# Autodesk Inventor assembly: 000 Ensamblaje hw_LM - BASIC
(part 3 of 4)
- [Flush]: UND_0201CR___ _________:69 ↔ UND_0201CR___ _________:70
- [Flush]: UND_0201CR___ _________:75 ↔ UND_0201CR___ _________:77
- [Flush]: UND_0201CR___ _________:76 ↔ UND_0201CR___ _________:77
- [Flush]: UND_0201CR___ _________:74 ↔ UND_0201CR___ _________:77
- [Flush]: UND_0201CR___ _________:73 ↔ UND_0201CR___ _________:75
- [Flush]: UND_0201CR___ _________:71 ↔ UND_0201CR___ _________:74
- [Flush]: UND_0201CR___ _________:72 ↔ UND_0201CR___ _________:75
- Flush:768: UND_0201CR___ _________:44 ↔ UND_0201CR___ _________:51
- Flush:769: UND_0201CR___ _________:43 ↔ UND_0201CR___ _________:76
- Flush:770: UND_0201CR___ _________:49 ↔ UND_0201CR___ _________:57
- Flush:771: UND_0201CR___ _________:60 ↔ UND_0201CR___ _________:67
- Flush:772: UND_0201CR___ _________:8 ↔ UND_0201CR___ _________:40
- Flush:773: UND_0201CR___ _________:69 ↔ UND_0201CR___ _________:77
- [Flush]: UND_0201CR___ _________:79 ↔ UND_0201CR___ _________:82
- [Flush]: UND_0201CR___ _________:81 ↔ UND_0201CR___ _________:82
- [Flush]: UND_0201CR___ _________:78 ↔ UND_0201CR___ _________:82
- [Flush]: UND_0201CR___ _________:80 ↔ UND_0201CR___ _________:83
- [Flush]: UND_0201CR___ _________:79 ↔ UND_0201CR___ _________:80
- [Flush]: UND_0201CR___ _________:86 ↔ UND_0201CR___ _________:89
- [Flush]: UND_0201CR___ _________:88 ↔ UND_0201CR___ _________:89
- [Flush]: UND_0201CR___ _________:85 ↔ UND_0201CR___ _________:89
- [Flush]: UND_0201CR___ _________:87 ↔ UND_0201CR___ _________:90
- [Flush]: UND_0201CR___ _________:86 ↔ UND_0201CR___ _________:87
- [Flush]: UND_0201CR___ _________:92 ↔ UND_0201CR___ _________:94
- [Flush]: UND_0201CR___ _________:93 ↔ UND_0201CR___ _________:94
- [Flush]: UND_0201CR___ _________:91 ↔ UND_0201CR___ _________:94
- [Flush]: UND_0201CR___ _________:90 ↔ UND_0201CR___ _________:92
- [Flush]: UND_0201CR___ _________:88 ↔ UND_0201CR___ _________:91
- [Flush]: UND_0201CR___ _________:89 ↔ UND_0201CR___ _________:92
- [Flush]: UND_0201CR___ _________:78 ↔ UND_0201CR___ _________:84
- [Flush]: UND_0201CR___ _________:86 ↔ UND_0201CR___ _________:94
- Flush:792: UND_0201CR___ _________:64 ↔ UND_0201CR___ _________:82
- Flush:793: UND_0201CR___ _________:60 ↔ UND_0201CR___ _________:88
- Flush:794: UND_0201CR___ _________:50 ↔ UND_0201CR___ _________:84
- Flush:795: UND_0201CR___ _________:65 ↔ UND_0201CR___ _________:90
- Flush:796: UND_0201CR___ _________:67 ↔ UND_0201CR___ _________:92
- Flush:797: UND_0201CR___ _________:57 ↔ UND_0201CR___ _________:70
- Flush:798: UND_0201CR___ _________:6 ↔ UND_0201CR___ _________:67
- Flush:799: UND_0201CR___ _________:39 ↔ UND_0201CR___ _________:83
- [Flush]: UND_0201CR___ _________:96 ↔ UND_0201CR___ _________:99
- [Flush]: UND_0201CR___ _________:98 ↔ UND_0201CR___ _________:99
- [Flush]: UND_0201CR___ _________:95 ↔ UND_0201CR___ _________:99
- [Flush]: UND_0201CR___ _________:97 ↔ UND_0201CR___ _________:100
- [Flush]: UND_0201CR___ _________:96 ↔ UND_0201CR___ _________:97
- [Flush]: UND_0201CR___ _________:103 ↔ UND_0201CR___ _________:106
- [Flush]: UND_0201CR___ _________:105 ↔ UND_0201CR___ _________:106
- [Flush]: UND_0201CR___ _________:102 ↔ UND_0201CR___ _________:106
- [Flush]: UND_0201CR___ _________:104 ↔ UND_0201CR___ _________:107
- [Flush]: UND_0201CR___ _________:103 ↔ UND_0201CR___ _________:104
- [Flush]: UND_0201CR___ _________:109 ↔ UND_0201CR___ _________:111
- [Flush]: UND_0201CR___ _________:110 ↔ UND_0201CR___ _________:111
- [Flush]: UND_0201CR___ _________:108 ↔ UND_0201CR___ _________:111
- [Flush]: UND_0201CR___ _________:107 ↔ UND_0201CR___ _________:109
- [Flush]: UND_0201CR___ _________:105 ↔ UND_0201CR___ _________:108
- [Flush]: UND_0201CR___ _________:106 ↔ UND_0201CR___ _________:109
- [Flush]: UND_0201CR___ _________:95 ↔ UND_0201CR___ _________:101
- [Flush]: UND_0201CR___ _________:103 ↔ UND_0201CR___ _________:111
- Flush:818: UND_0201CR___ _________:92 ↔ UND_0201CR___ _________:108
- Flush:819: UND_0201CR___ _________:81 ↔ UND_0201CR___ _________:101
- [Flush]: UND_0201CR___ _________:112 ↔ UND_0201CR___ _________:113
- Angle:201 (0 deg): AQ24CANFD-02HTG:8 ↔ UND_0201CR___ _________:112
- Angle:202 (0 deg): UND_0201CR___ _________:112 ↔ UND_0201CR___ _________:114
- Angle:203 (0 deg): UND_0201CR___ _________:113 ↔ UND_0201CR___ _________:114
- Flush:821: UND_0201CR___ _________:113 ↔ UND_0201CR___ _________:114
- Flush:822: UND_0201CR___ _________:112 ↔ UND_0201CR___ _________:113
- Flush:823: UND_0201CR___ _________:84 ↔ UND_0201CR___ _________:113
- [Flush]: UND_0201CR___ _________:115 ↔ UND_0201CR___ _________:116
- [Angle] (0 deg): UND_0201CR___ _________:115 ↔ UND_0201CR___ _________:117
- [Angle] (0 deg): UND_0201CR___ _________:116 ↔ UND_0201CR___ _________:117
- [Flush]: UND_0201CR___ _________:116 ↔ UND_0201CR___ _________:117
- [Flush]: UND_0201CR___ _________:115 ↔ UND_0201CR___ _________:116
- [Flush]: UND_0201CR___ _________:118 ↔ UND_0201CR___ _________:119
- [Angle] (0 deg): UND_0201CR___ _________:118 ↔ UND_0201CR___ _________:120
- [Angle] (0 deg): UND_0201CR___ _________:119 ↔ UND_0201CR___ _________:120
- [Flush]: UND_0201CR___ _________:119 ↔ UND_0201CR___ _________:120
- [Flush]: UND_0201CR___ _________:118 ↔ UND_0201CR___ _________:119
- Flush:830: UND_0201CR___ _________:114 ↔ UND_0201CR___ _________:117
- Flush:831: UND_0201CR___ _________:112 ↔ UND_0201CR___ _________:118
- Flush:832: UND_0201CR___ _________:113 ↔ UND_0201CR___ _________:116
- Flush:833: UND_0201CR___ _________:115 ↔ UND_0201CR___ _________:118
- [Flush]: UND_0201CR___ _________:121 ↔ UND_0201CR___ _________:122
- [Angle] (0 deg): UND_0201CR___ _________:121 ↔ UND_0201CR___ _________:123
- [Angle] (0 deg): UND_0201CR___ _________:122 ↔ UND_0201CR___ _________:123
- [Flush]: UND_0201CR___ _________:122 ↔ UND_0201CR___ _________:123
- [Flush]: UND_0201CR___ _________:121 ↔ UND_0201CR___ _________:122
- [Flush]: UND_0201CR___ _________:124 ↔ UND_0201CR___ _________:125
- [Angle] (0 deg): UND_0201CR___ _________:124 ↔ UND_0201CR___ _________:126
- [Angle] (0 deg): UND_0201CR___ _________:125 ↔ UND_0201CR___ _________:126
- [Flush]: UND_0201CR___ _________:125 ↔ UND_0201CR___ _________:126
- [Flush]: UND_0201CR___ _________:124 ↔ UND_0201CR___ _________:125
- [Flush]: UND_0201CR___ _________:127 ↔ UND_0201CR___ _________:128
- [Angle] (0 deg): UND_0201CR___ _________:127 ↔ UND_0201CR___ _________:129
- [Angle] (0 deg): UND_0201CR___ _________:128 ↔ UND_0201CR___ _________:129
- [Flush]: UND_0201CR___ _________:128 ↔ UND_0201CR___ _________:129
- [Flush]: UND_0201CR___ _________:127 ↔ UND_0201CR___ _________:128
- [Flush]: UND_0201CR___ _________:123 ↔ UND_0201CR___ _________:126
- [Flush]: UND_0201CR___ _________:121 ↔ UND_0201CR___ _________:127
- [Flush]: UND_0201CR___ _________:122 ↔ UND_0201CR___ _________:125
- [Flush]: UND_0201CR___ _________:124 ↔ UND_0201CR___ _________:127
- [Flush]: UND_0201CR___ _________:130 ↔ UND_0201CR___ _________:131
- [Angle] (0 deg): UND_0201CR___ _________:130 ↔ UND_0201CR___ _________:132
- [Angle] (0 deg): UND_0201CR___ _________:131 ↔ UND_0201CR___ _________:132
- [Flush]: UND_0201CR___ _________:131 ↔ UND_0201CR___ _________:132
- [Flush]: UND_0201CR___ _________:130 ↔ UND_0201CR___ _________:131
- [Flush]: UND_0201CR___ _________:133 ↔ UND_0201CR___ _________:134
- [Angle] (0 deg): UND_0201CR___ _________:133 ↔ UND_0201CR___ _________:135
- [Angle] (0 deg): UND_0201CR___ _________:134 ↔ UND_0201CR___ _________:135
- [Flush]: UND_0201CR___ _________:134 ↔ UND_0201CR___ _________:135
- [Flush]: UND_0201CR___ _________:133 ↔ UND_0201CR___ _________:134
- [Flush]: UND_0201CR___ _________:136 ↔ UND_0201CR___ _________:137
- [Angle] (0 deg): UND_0201CR___ _________:136 ↔ UND_0201CR___ _________:138
- [Angle] (0 deg): UND_0201CR___ _________:137 ↔ UND_0201CR___ _________:138
- [Flush]: UND_0201CR___ _________:137 ↔ UND_0201CR___ _________:138
- [Flush]: UND_0201CR___ _________:136 ↔ UND_0201CR___ _________:137
- [Flush]: UND_0201CR___ _________:132 ↔ UND_0201CR___ _________:135
- [Flush]: UND_0201CR___ _________:130 ↔ UND_0201CR___ _________:136
- [Flush]: UND_0201CR___ _________:131 ↔ UND_0201CR___ _________:134
- [Flush]: UND_0201CR___ _________:133 ↔ UND_0201CR___ _________:136
- Flush:860: UND_0201CR___ _________:84 ↔ UND_0201CR___ _________:129
- Flush:861: UND_0201CR___ _________:122 ↔ UND_0201CR___ _________:132
- Flush:862: UND_0201CR___ _________:125 ↔ UND_0201CR___ _________:133
- [Flush]: UND_0201CR___ _________:139 ↔ UND_0201CR___ _________:140
- [Angle] (0 deg): UND_0201CR___ _________:139 ↔ UND_0201CR___ _________:141
- [Angle] (0 deg): UND_0201CR___ _________:140 ↔ UND_0201CR___ _________:141
- [Flush]: UND_0201CR___ _________:140 ↔ UND_0201CR___ _________:141
- [Flush]: UND_0201CR___ _________:139 ↔ UND_0201CR___ _________:140
- [Flush]: UND_0201CR___ _________:142 ↔ UND_0201CR___ _________:143
- [Angle] (0 deg): UND_0201CR___ _________:142 ↔ UND_0201CR___ _________:144
- [Angle] (0 deg): UND_0201CR___ _________:143 ↔ UND_0201CR___ _________:144
- [Flush]: UND_0201CR___ _________:143 ↔ UND_0201CR___ _________:144
- [Flush]: UND_0201CR___ _________:142 ↔ UND_0201CR___ _________:143
- [Flush]: UND_0201CR___ _________:145 ↔ UND_0201CR___ _________:146
- [Angle] (0 deg): UND_0201CR___ _________:145 ↔ UND_0201CR___ _________:147
- [Angle] (0 deg): UND_0201CR___ _________:146 ↔ UND_0201CR___ _________:147
- [Flush]: UND_0201CR___ _________:146 ↔ UND_0201CR___ _________:147
- [Flush]: UND_0201CR___ _________:145 ↔ UND_0201CR___ _________:146
- [Flush]: UND_0201CR___ _________:141 ↔ UND_0201CR___ _________:144
- [Flush]: UND_0201CR___ _________:139 ↔ UND_0201CR___ _________:145
- [Flush]: UND_0201CR___ _________:140 ↔ UND_0201CR___ _________:143
- [Flush]: UND_0201CR___ _________:142 ↔ UND_0201CR___ _________:145
- [Flush]: UND_0201CR___ _________:148 ↔ UND_0201CR___ _________:149
- [Angle] (0 deg): UND_0201CR___ _________:148 ↔ UND_0201CR___ _________:150
- [Angle] (0 deg): UND_0201CR___ _________:149 ↔ UND_0201CR___ _________:150
- [Flush]: UND_0201CR___ _________:149 ↔ UND_0201CR___ _________:150
- [Flush]: UND_0201CR___ _________:148 ↔ UND_0201CR___ _________:149
- [Flush]: UND_0201CR___ _________:151 ↔ UND_0201CR___ _________:152
- [Angle] (0 deg): UND_0201CR___ _________:151 ↔ UND_0201CR___ _________:153
- [Angle] (0 deg): UND_0201CR___ _________:152 ↔ UND_0201CR___ _________:153
- [Flush]: UND_0201CR___ _________:152 ↔ UND_0201CR___ _________:153
- [Flush]: UND_0201CR___ _________:151 ↔ UND_0201CR___ _________:152
- [Flush]: UND_0201CR___ _________:154 ↔ UND_0201CR___ _________:155
- [Angle] (0 deg): UND_0201CR___ _________:154 ↔ UND_0201CR___ _________:156
- [Angle] (0 deg): UND_0201CR___ _________:155 ↔ UND_0201CR___ _________:156
- [Flush]: UND_0201CR___ _________:155 ↔ UND_0201CR___ _________:156
- [Flush]: UND_0201CR___ _________:154 ↔ UND_0201CR___ _________:155
- [Flush]: UND_0201CR___ _________:150 ↔ UND_0201CR___ _________:153
- [Flush]: UND_0201CR___ _________:148 ↔ UND_0201CR___ _________:154
- [Flush]: UND_0201CR___ _________:149 ↔ UND_0201CR___ _________:152
- [Flush]: UND_0201CR___ _________:151 ↔ UND_0201CR___ _________:154
- Flush:889: UND_0201CR___ _________:84 ↔ UND_0201CR___ _________:149
- Flush:890: UND_0201CR___ _________:131 ↔ UND_0201CR___ _________:139
- Flush:891: UND_0201CR___ _________:144 ↔ UND_0201CR___ _________:148
- [Flush]: UND_0201CR___ _________:157 ↔ UND_0201CR___ _________:158
- [Angle] (0 deg): UND_0201CR___ _________:157 ↔ UND_0201CR___ _________:159
- [Angle] (0 deg): UND_0201CR___ _________:158 ↔ UND_0201CR___ _________:159
- [Flush]: UND_0201CR___ _________:158 ↔ UND_0201CR___ _________:159
- [Flush]: UND_0201CR___ _________:157 ↔ UND_0201CR___ _________:158
- [Flush]: UND_0201CR___ _________:160 ↔ UND_0201CR___ _________:161
- [Angle] (0 deg): UND_0201CR___ _________:160 ↔ UND_0201CR___ _________:162
- [Angle] (0 deg): UND_0201CR___ _________:161 ↔ UND_0201CR___ _________:162
- [Flush]: UND_0201CR___ _________:161 ↔ UND_0201CR___ _________:162
- [Flush]: UND_0201CR___ _________:160 ↔ UND_0201CR___ _________:161
- [Flush]: UND_0201CR___ _________:163 ↔ UND_0201CR___ _________:164
- [Angle] (0 deg): UND_0201CR___ _________:163 ↔ UND_0201CR___ _________:165
- [Angle] (0 deg): UND_0201CR___ _________:164 ↔ UND_0201CR___ _________:165
- [Flush]: UND_0201CR___ _________:164 ↔ UND_0201CR___ _________:165
- [Flush]: UND_0201CR___ _________:163 ↔ UND_0201CR___ _________:164
- [Flush]: UND_0201CR___ _________:159 ↔ UND_0201CR___ _________:162
- [Flush]: UND_0201CR___ _________:157 ↔ UND_0201CR___ _________:163
- [Flush]: UND_0201CR___ _________:158 ↔ UND_0201CR___ _________:161
- [Flush]: UND_0201CR___ _________:160 ↔ UND_0201CR___ _________:163
- [Flush]: UND_0201CR___ _________:166 ↔ UND_0201CR___ _________:167
- [Angle] (0 deg): UND_0201CR___ _________:166 ↔ UND_0201CR___ _________:168
- [Angle] (0 deg): UND_0201CR___ _________:167 ↔ UND_0201CR___ _________:168
- [Flush]: UND_0201CR___ _________:167 ↔ UND_0201CR___ _________:168
- [Flush]: UND_0201CR___ _________:166 ↔ UND_0201CR___ _________:167
- [Flush]: UND_0201CR___ _________:169 ↔ UND_0201CR___ _________:170
- [Angle] (0 deg): UND_0201CR___ _________:169 ↔ UND_0201CR___ _________:171
- [Angle] (0 deg): UND_0201CR___ _________:170 ↔ UND_0201CR___ _________:171
- [Flush]: UND_0201CR___ _________:170 ↔ UND_0201CR___ _________:171
- [Flush]: UND_0201CR___ _________:169 ↔ UND_0201CR___ _________:170
- [Flush]: UND_0201CR___ _________:172 ↔ UND_0201CR___ _________:173
- [Angle] (0 deg): UND_0201CR___ _________:172 ↔ UND_0201CR___ _________:174
- [Angle] (0 deg): UND_0201CR___ _________:173 ↔ UND_0201CR___ _________:174
- [Flush]: UND_0201CR___ _________:173 ↔ UND_0201CR___ _________:174
- [Flush]: UND_0201CR___ _________:172 ↔ UND_0201CR___ _________:173
- [Flush]: UND_0201CR___ _________:168 ↔ UND_0201CR___ _________:171
- [Flush]: UND_0201CR___ _________:166 ↔ UND_0201CR___ _________:172
- [Flush]: UND_0201CR___ _________:167 ↔ UND_0201CR___ _________:170
- [Flush]: UND_0201CR___ _________:169 ↔ UND_0201CR___ _________:172
- Flush:918: UND_0201CR___ _________:144 ↔ UND_0201CR___ _________:159
- Flush:919: UND_0201CR___ _________:159 ↔ UND_0201CR___ _________:168
- Flush:920: UND_0201CR___ _________:146 ↔ UND_0201CR___ _________:167
- Flush:921: UND_0201CR___ _________:162 ↔ UND_0201CR___ _________:171
- [Flush]: UND_0201CR___ _________:175 ↔ UND_0201CR___ _________:176
- [Angle] (0 deg): UND_0201CR___ _________:175 ↔ UND_0201CR___ _________:177
- [Angle] (0 deg): UND_0201CR___ _________:176 ↔ UND_0201CR___ _________:177
- [Flush]: UND_0201CR___ _________:176 ↔ UND_0201CR___ _________:177
- [Flush]: UND_0201CR___ _________:175 ↔ UND_0201CR___ _________:176
- [Flush]: UND_0201CR___ _________:178 ↔ UND_0201CR___ _________:179
- [Angle] (0 deg): UND_0201CR___ _________:178 ↔ UND_0201CR___ _________:180
- [Angle] (0 deg): UND_0201CR___ _________:179 ↔ UND_0201CR___ _________:180
- [Flush]: UND_0201CR___ _________:179 ↔ UND_0201CR___ _________:180
- [Flush]: UND_0201CR___ _________:178 ↔ UND_0201CR___ _________:179
- [Flush]: UND_0201CR___ _________:181 ↔ UND_0201CR___ _________:182
- [Angle] (0 deg): UND_0201CR___ _________:181 ↔ UND_0201CR___ _________:183
- [Angle] (0 deg): UND_0201CR___ _________:182 ↔ UND_0201CR___ _________:183
- [Flush]: UND_0201CR___ _________:182 ↔ UND_0201CR___ _________:183
- [Flush]: UND_0201CR___ _________:181 ↔ UND_0201CR___ _________:182
- [Flush]: UND_0201CR___ _________:177 ↔ UND_0201CR___ _________:180
- [Flush]: UND_0201CR___ _________:175 ↔ UND_0201CR___ _________:181
- [Flush]: UND_0201CR___ _________:176 ↔ UND_0201CR___ _________:179
- [Flush]: UND_0201CR___ _________:178 ↔ UND_0201CR___ _________:181
- [Flush]: UND_0201CR___ _________:184 ↔ UND_0201CR___ _________:185
- [Angle] (0 deg): UND_0201CR___ _________:184 ↔ UND_0201CR___ _________:186
- [Angle] (0 deg): UND_0201CR___ _________:185 ↔ UND_0201CR___ _________:186
- [Flush]: UND_0201CR___ _________:185 ↔ UND_0201CR___ _________:186
- [Flush]: UND_0201CR___ _________:184 ↔ UND_0201CR___ _________:185
- [Flush]: UND_0201CR___ _________:187 ↔ UND_0201CR___ _________:188
- [Angle] (0 deg): UND_0201CR___ _________:187 ↔ UND_0201CR___ _________:189
- [Angle] (0 deg): UND_0201CR___ _________:188 ↔ UND_0201CR___ _________:189
- [Flush]: UND_0201CR___ _________:188 ↔ UND_0201CR___ _________:189
- [Flush]: UND_0201CR___ _________:187 ↔ UND_0201CR___ _________:188
- [Flush]: UND_0201CR___ _________:190 ↔ UND_0201CR___ _________:191
- [Angle] (0 deg): UND_0201CR___ _________:190 ↔ UND_0201CR___ _________:192
- [Angle] (0 deg): UND_0201CR___ _________:191 ↔ UND_0201CR___ _________:192
- [Flush]: UND_0201CR___ _________:191 ↔ UND_0201CR___ _________:192
- [Flush]: UND_0201CR___ _________:190 ↔ UND_0201CR___ _________:191
- [Flush]: UND_0201CR___ _________:186 ↔ UND_0201CR___ _________:189
- [Flush]: UND_0201CR___ _________:184 ↔ UND_0201CR___ _________:190
- [Flush]: UND_0201CR___ _________:185 ↔ UND_0201CR___ _________:188
- [Flush]: UND_0201CR___ _________:187 ↔ UND_0201CR___ _________:190
- Flush:948: UND_0201CR___ _________:176 ↔ UND_0201CR___ _________:185
- Flush:949: UND_0201CR___ _________:167 ↔ UND_0201CR___ _________:176
- Flush:950: UND_0201CR___ _________:175 ↔ UND_0201CR___ _________:191
- Flush:951: UND_0201CR___ _________:180 ↔ UND_0201CR___ _________:187
- Flush:952: UND_0201CR___ _________:171 ↔ UND_0201CR___ _________:178
- Flush:953: UND_0201CR___ _________:170 ↔ UND_0201CR___ _________:182
- [Flush]: UND_0201CR___ _________:193 ↔ UND_0201CR___ _________:194
- [Angle] (0 deg): UND_0201CR___ _________:193 ↔ UND_0201CR___ _________:195
- [Angle] (0 deg): UND_0201CR___ _________:194 ↔ UND_0201CR___ _________:195
- [Flush]: UND_0201CR___ _________:194 ↔ UND_0201CR___ _________:195
- [Flush]: UND_0201CR___ _________:193 ↔ UND_0201CR___ _________:194
- [Flush]: UND_0201CR___ _________:196 ↔ UND_0201CR___ _________:197
- [Angle] (0 deg): UND_0201CR___ _________:196 ↔ UND_0201CR___ _________:198
- [Angle] (0 deg): UND_0201CR___ _________:197 ↔ UND_0201CR___ _________:198
- [Flush]: UND_0201CR___ _________:197 ↔ UND_0201CR___ _________:198
- [Flush]: UND_0201CR___ _________:196 ↔ UND_0201CR___ _________:197
- [Flush]: UND_0201CR___ _________:199 ↔ UND_0201CR___ _________:200
- [Angle] (0 deg): UND_0201CR___ _________:199 ↔ UND_0201CR___ _________:201
- [Angle] (0 deg): UND_0201CR___ _________:200 ↔ UND_0201CR___ _________:201
- [Flush]: UND_0201CR___ _________:200 ↔ UND_0201CR___ _________:201
- [Flush]: UND_0201CR___ _________:199 ↔ UND_0201CR___ _________:200
- [Flush]: UND_0201CR___ _________:195 ↔ UND_0201CR___ _________:198
- [Flush]: UND_0201CR___ _________:193 ↔ UND_0201CR___ _________:199
- [Flush]: UND_0201CR___ _________:194 ↔ UND_0201CR___ _________:197
- [Flush]: UND_0201CR___ _________:196 ↔ UND_0201CR___ _________:199
- [Angle] (0 deg): UND_0201CR___ _________:202 ↔ UND_0201CR___ _________:203
- [Flush]: UND_0201CR___ _________:204 ↔ UND_0201CR___ _________:205
- [Angle] (0 deg): UND_0201CR___ _________:204 ↔ UND_0201CR___ _________:206
- [Angle] (0 deg): UND_0201CR___ _________:205 ↔ UND_0201CR___ _________:206
- [Flush]: UND_0201CR___ _________:205 ↔ UND_0201CR___ _________:206
- [Flush]: UND_0201CR___ _________:204 ↔ UND_0201CR___ _________:205
- [Flush]: UND_0201CR___ _________:202 ↔ UND_0201CR___ _________:204
- [Flush]: UND_0201CR___ _________:198 ↔ UND_0201CR___ _________:202
- [Flush]: UND_0201CR___ _________:197 ↔ UND_0201CR___ _________:205
- Flush:973: UND_0201CR___ _________:167 ↔ UND_0201CR___ _________:193
- Flush:974: UND_0201CR___ _________:178 ↔ UND_0201CR___ _________:194
- Flush:975: UND_0201CR___ _________:195 ↔ UND_0201CR___ _________:202
- Flush:976: UND_0201CR___ _________:182 ↔ UND_0201CR___ _________:193
- [Angle] (0 deg): UND_0201CR___ _________:207 ↔ UND_0201CR___ _________:208
- [Flush]: UND_0201CR___ _________:209 ↔ UND_0201CR___ _________:210
- [Angle] (0 deg): UND_0201CR___ _________:209 ↔ UND_0201CR___ _________:211
- [Angle] (0 deg): UND_0201CR___ _________:210 ↔ UND_0201CR___ _________:211
- [Flush]: UND_0201CR___ _________:210 ↔ UND_0201CR___ _________:211
- [Flush]: UND_0201CR___ _________:209 ↔ UND_0201CR___ _________:210
- [Flush]: UND_0201CR___ _________:207 ↔ UND_0201CR___ _________:209
- [Flush]: UND_0201CR___ _________:212 ↔ UND_0201CR___ _________:213
- [Angle] (0 deg): UND_0201CR___ _________:212 ↔ UND_0201CR___ _________:214
- [Angle] (0 deg): UND_0201CR___ _________:213 ↔ UND_0201CR___ _________:214
- [Flush]: UND_0201CR___ _________:213 ↔ UND_0201CR___ _________:214
- [Flush]: UND_0201CR___ _________:212 ↔ UND_0201CR___ _________:213
- [Flush]: UND_0201CR___ _________:215 ↔ UND_0201CR___ _________:216
- [Angle] (0 deg): UND_0201CR___ _________:215 ↔ UND_0201CR___ _________:217
- [Angle] (0 deg): UND_0201CR___ _________:216 ↔ UND_0201CR___ _________:217
- [Flush]: UND_0201CR___ _________:216 ↔ UND_0201CR___ _________:217
- [Flush]: UND_0201CR___ _________:215 ↔ UND_0201CR___ _________:216
- [Flush]: UND_0201CR___ _________:218 ↔ UND_0201CR___ _________:219
- [Angle] (0 deg): UND_0201CR___ _________:218 ↔ UND_0201CR___ _________:220
- [Angle] (0 deg): UND_0201CR___ _________:219 ↔ UND_0201CR___ _________:220
- [Flush]: UND_0201CR___ _________:219 ↔ UND_0201CR___ _________:220
- [Flush]: UND_0201CR___ _________:218 ↔ UND_0201CR___ _________:219
- [Flush]: UND_0201CR___ _________:214 ↔ UND_0201CR___ _________:217
- [Flush]: UND_0201CR___ _________:212 ↔ UND_0201CR___ _________:218
- [Flush]: UND_0201CR___ _________:213 ↔ UND_0201CR___ _________:216
- [Flush]: UND_0201CR___ _________:215 ↔ UND_0201CR___ _________:218
- [Flush]: UND_0201CR___ _________:207 ↔ UND_0201CR___ _________:213
- [Flush]: UND_0201CR___ _________:210 ↔ UND_0201CR___ _________:212
- Flush:996: UND_0201CR___ _________:201 ↔ UND_0201CR___ _________:213
- Flush:997: UND_0201CR___ _________:198 ↔ UND_0201CR___ _________:207
- Flush:998: UND_0201CR___ _________:178 ↔ UND_0201CR___ _________:218
- [Angle] (0 deg): UND_0201CR___ _________:221 ↔ UND_0201CR___ _________:222
- [Flush]: UND_0201CR___ _________:223 ↔ UND_0201CR___ _________:224
- [Angle] (0 deg): UND_0201CR___ _________:223 ↔ UND_0201CR___ _________:225
- [Angle] (0 deg): UND_0201CR___ _________:224 ↔ UND_0201CR___ _________:225
- [Flush]: UND_0201CR___ _________:224 ↔ UND_0201CR___ _________:225
- [Flush]: UND_0201CR___ _________:223 ↔ UND_0201CR___ _________:224
- [Flush]: UND_0201CR___ _________:226 ↔ UND_0201CR___ _________:227
- [Angle] (0 deg): UND_0201CR___ _________:226 ↔ UND_0201CR___ _________:228
- [Angle] (0 deg): UND_0201CR___ _________:227 ↔ UND_0201CR___ _________:228
- [Flush]: UND_0201CR___ _________:227 ↔ UND_0201CR___ _________:228
- [Flush]: UND_0201CR___ _________:226 ↔ UND_0201CR___ _________:227
- [Flush]: UND_0201CR___ _________:222 ↔ UND_0201CR___ _________:225
- [Flush]: UND_0201CR___ _________:221 ↔ UND_0201CR___ _________:226
- [Flush]: UND_0201CR___ _________:223 ↔ UND_0201CR___ _________:226
- Flush:1008: UND_0201CR___ _________:220 ↔ UND_0201CR___ _________:221
- Flush:1009: UND_0201CR___ _________:208 ↔ UND_0201CR___ _________:223
- [Angle] (0 deg): UND_0201CR___ _________:229 ↔ UND_0201CR___ _________:230
- [Flush]: UND_0201CR___ _________:231 ↔ UND_0201CR___ _________:232
- [Angle] (0 deg): UND_0201CR___ _________:231 ↔ UND_0201CR___ _________:233
- [Angle] (0 deg): UND_0201CR___ _________:232 ↔ UND_0201CR___ _________:233
- [Flush]: UND_0201CR___ _________:232 ↔ UND_0201CR___ _________:233
- [Flush]: UND_0201CR___ _________:231 ↔ UND_0201CR___ _________:232
- [Flush]: UND_0201CR___ _________:234 ↔ UND_0201CR___ _________:235
- [Angle] (0 deg): UND_0201CR___ _________:234 ↔ UND_0201CR___ _________:236
- [Angle] (0 deg): UND_0201CR___ _________:235 ↔ UND_0201CR___ _________:236
- [Flush]: UND_0201CR___ _________:235 ↔ UND_0201CR___ _________:236
- [Flush]: UND_0201CR___ _________:234 ↔ UND_0201CR___ _________:235
- [Flush]: UND_0201CR___ _________:230 ↔ UND_0201CR___ _________:233
- [Flush]: UND_0201CR___ _________:229 ↔ UND_0201CR___ _________:234
- [Flush]: UND_0201CR___ _________:231 ↔ UND_0201CR___ _________:234
- [Angle] (0 deg): UND_0201CR___ _________:237 ↔ UND_0201CR___ _________:238
- [Flush]: UND_0201CR___ _________:239 ↔ UND_0201CR___ _________:240
- [Angle] (0 deg): UND_0201CR___ _________:239 ↔ UND_0201CR___ _________:241
- [Angle] (0 deg): UND_0201CR___ _________:240 ↔ UND_0201CR___ _________:241
- [Flush]: UND_0201CR___ _________:240 ↔ UND_0201CR___ _________:241
- [Flush]: UND_0201CR___ _________:239 ↔ UND_0201CR___ _________:240
- [Flush]: UND_0201CR___ _________:242 ↔ UND_0201CR___ _________:243
- [Angle] (0 deg): UND_0201CR___ _________:242 ↔ UND_0201CR___ _________:244
- [Angle] (0 deg): UND_0201CR___ _________:243 ↔ UND_0201CR___ _________:244
- [Flush]: UND_0201CR___ _________:243 ↔ UND_0201CR___ _________:244
- [Flush]: UND_0201CR___ _________:242 ↔ UND_0201CR___ _________:243
- [Flush]: UND_0201CR___ _________:238 ↔ UND_0201CR___ _________:241
- [Flush]: UND_0201CR___ _________:237 ↔ UND_0201CR___ _________:242
- [Flush]: UND_0201CR___ _________:239 ↔ UND_0201CR___ _________:242
- Flush:1028: UND_0201CR___ _________:236 ↔ UND_0201CR___ _________:238
- Flush:1029: UND_0201CR___ _________:226 ↔ UND_0201CR___ _________:229
- Flush:1030: UND_0201CR___ _________:232 ↔ UND_0201CR___ _________:240
- Flush:1031: UND_0201CR___ _________:221 ↔ UND_0201CR___ _________:233
- Flush:1032: UND_0201CR___ _________:225 ↔ UND_0201CR___ _________:242
- Flush:1033: UND_0201CR___ _________:230 ↔ UND_0201CR___ _________:237
- Flush:1034: UND_0201CR___ _________:231 ↔ UND_0201CR___ _________:240
- Flush:1035: UND_0201CR___ _________:84 ↔ UND_0201CR___ _________:237
- Flush:1036: UND_0201CR___ _________:165 ↔ UND_0201CR___ _________:236
- [Flush]: UND_0201CR___ _________:250 ↔ UND_0201CR___ _________:251
- [Angle] (0 deg): UND_0201CR___ _________:250 ↔ UND_0201CR___ _________:252
- [Angle] (0 deg): UND_0201CR___ _________:251 ↔ UND_0201CR___ _________:252
- [Flush]: UND_0201CR___ _________:251 ↔ UND_0201CR___ _________:252
- [Flush]: UND_0201CR___ _________:250 ↔ UND_0201CR___ _________:251
- [Angle] (0 deg): UND_0201CR___ _________:261 ↔ UND_0201CR___ _________:262
- [Flush]: UND_0201CR___ _________:266 ↔ UND_0201CR___ _________:267
- [Angle] (0 deg): UND_0201CR___ _________:266 ↔ UND_0201CR___ _________:268
- [Angle] (0 deg): UND_0201CR___ _________:267 ↔ UND_0201CR___ _________:268
- [Flush]: UND_0201CR___ _________:267 ↔ UND_0201CR___ _________:268
- [Flush]: UND_0201CR___ _________:266 ↔ UND_0201CR___ _________:267
- [Flush]: UND_0201CR___ _________:261 ↔ UND_0201CR___ _________:266
- Flush:1069: UND_0201CR___ _________:229 ↔ UND_0201CR___ _________:266
- Flush:1070: RES-1.6K_1%_0402:332 ↔ RES-1.6K_1%_0402:333
- Flush:1071: RES-1.6K_1%_0402:334 ↔ RES-1.6K_1%_0402:335
- Flush:1072: RES-1.6K_1%_0402:335 ↔ RES-1.6K_1%_0402:259
- Flush:1073: RES-1.6K_1%_0402:333 ↔ RES-1.6K_1%_0402:259
- Flush:1074: RES-1.6K_1%_0402:336 ↔ RES-1.6K_1%_0402:339
- Flush:1075: RES-1.6K_1%_0402:333 ↔ RES-1.6K_1%_0402:337
- [Flush]: RES-1.6K_1%_0402:340 ↔ RES-1.6K_1%_0402:343
- Flush:1077: RES-1.6K_1%_0402:338 ↔ RES-1.6K_1%_0402:339
- Flush:1078: RES-1.6K_1%_0402:332 ↔ RES-1.6K_1%_0402:337
- Flush:1079: RES-1.6K_1%_0402:337 ↔ RES-1.6K_1%_0402:338
- Flush:1080: RES-1.6K_1%_0402:338 ↔ RES-1.6K_1%_0402:340
- Flush:1081: RES-1.6K_1%_0402:341 ↔ RES-1.6K_1%_0402:342
- Flush:1082: RES-1.6K_1%_0402:340 ↔ RES-1.6K_1%_0402:343
- Flush:1083: RES-1.6K_1%_0402:341 ↔ RES-1.6K_1%_0402:342
- [Flush]: RES-1.6K_1%_0402:344 ↔ RES-1.6K_1%_0402:345
- [Flush]: RES-1.6K_1%_0402:344 ↔ RES-1.6K_1%_0402:345
- [Flush]: RES-1.6K_1%_0402:346 ↔ RES-1.6K_1%_0402:347
- [Flush]: RES-1.6K_1%_0402:346 ↔ RES-1.6K_1%_0402:347
- [Flush]: RES-1.6K_1%_0402:348 ↔ RES-1.6K_1%_0402:349
- [Flush]: RES-1.6K_1%_0402:348 ↔ RES-1.6K_1%_0402:349
- Flush:1090: RES-1.6K_1%_0402:345 ↔ RES-1.6K_1%_0402:346
- Flush:1091: RES-1.6K_1%_0402:341 ↔ RES-1.6K_1%_0402:344
- Flush:1092: RES-1.6K_1%_0402:347 ↔ RES-1.6K_1%_0402:259
- Flush:1093: RES-1.6K_1%_0402:345 ↔ RES-1.6K_1%_0402:296
- [Flush]: RES-1.6K_1%_0402:350 ↔ RES-1.6K_1%_0402:351
- [Flush]: RES-1.6K_1%_0402:350 ↔ RES-1.6K_1%_0402:351
- [Flush]: RES-1.6K_1%_0402:352 ↔ RES-1.6K_1%_0402:353
- [Flush]: RES-1.6K_1%_0402:352 ↔ RES-1.6K_1%_0402:353
- [Flush]: RES-1.6K_1%_0402:351 ↔ RES-1.6K_1%_0402:352
- Flush:1099: RES-1.6K_1%_0402:348 ↔ RES-1.6K_1%_0402:352
- Flush:1100: RES-1.6K_1%_0402:335 ↔ RES-1.6K_1%_0402:348
- Flush:1101: C0603C103K1RECAUTO:40 ↔ C0603C103K1RECAUTO:48
- Flush:1102: C0603C103K1RECAUTO:47 ↔ C0603C103K1RECAUTO:48
- Flush:1103: C0603C103K1RECAUTO:46 ↔ C0603C103K1RECAUTO:47
- Flush:1104: C0603C103K1RECAUTO:45 ↔ C0603C103K1RECAUTO:46
- [Flush]: C0603C103K1RECAUTO:49 ↔ C0603C103K1RECAUTO:50
- Flush:1106: C0603C103K1RECAUTO:40 ↔ C0603C103K1RECAUTO:49
- [Flush]: C0603C103K1RECAUTO:51 ↔ C0603C103K1RECAUTO:52
- Flush:1108: C0603C103K1RECAUTO:50 ↔ C0603C103K1RECAUTO:51
- Angle:304 (0 deg): TPS7A5301QRGRRQ1:2 ↔ C0603C103K1RECAUTO:52
- Angle:305 (0 deg): C0603C103K1RECAUTO:50 ↔ C0603C103K1RECAUTO:52
- Angle:306 (0 deg): C0603C103K1RECAUTO:49 ↔ C0603C103K1RECAUTO:50
- Flush:1109: RES-1.6K_1%_0402:355 ↔ RES-1.6K_1%_0402:357
- Flush:1110: RES-1.6K_1%_0402:354 ↔ RES-1.6K_1%_0402:355
- Flush:1111: RES-1.6K_1%_0402:354 ↔ RES-1.6K_1%_0402:356
- Flush:1112: RES-1.6K_1%_0402:347 ↔ RES-1.6K_1%_0402:357
- [Flush]: RES-1.6K_1%_0402:358 ↔ RES-1.6K_1%_0402:359
- Flush:1116: RES-1.6K_1%_0402:346 ↔ RES-1.6K_1%_0402:359
- Flush:1117: RES-1.6K_1%_0402:347 ↔ RES-1.6K_1%_0402:361
- Flush:1118: RES-1.6K_1%_0402:360 ↔ RES-1.6K_1%_0402:361
- Flush:1119: RES-1.6K_1%_0402:348 ↔ RES-1.6K_1%_0402:360
- [Flush]: RES-1.6K_1%_0402:363 ↔ RES-1.6K_1%_0402:364
- [Flush]: RES-1.6K_1%_0402:362 ↔ RES-1.6K_1%_0402:363
- [Flush]: RES-1.6K_1%_0402:366 ↔ RES-1.6K_1%_0402:367
- [Flush]: RES-1.6K_1%_0402:365 ↔ RES-1.6K_1%_0402:366
- Flush:1124: RES-1.6K_1%_0402:364 ↔ RES-1.6K_1%_0402:366
- Flush:1125: RES-1.6K_1%_0402:362 ↔ RES-1.6K_1%_0402:367
- Flush:1126: RES-1.6K_1%_0402:363 ↔ RES-1.6K_1%_0402:366
- Flush:1127: RES-1.6K_1%_0402:364 ↔ RES-1.6K_1%_0402:365
- Flush:1128: RES-1.6K_1%_0402:346 ↔ RES-1.6K_1%_0402:362
- Flush:1129: C0603C103K1RECAUTO:40 ↔ C0603C103K1RECAUTO:53
- Flush:1130: UND_0201CR___ _________:36 ↔ UND_0201CR___ _________:269
- [Flush]: RES-1.6K_1%_0402:369 ↔ RES-1.6K_1%_0402:370
- Flush:1132: RES-1.6K_1%_0402:343 ↔ RES-1.6K_1%_0402:368
- Flush:1133: RES-1.6K_1%_0402:368 ↔ RES-1.6K_1%_0402:370
- Flush:1134: RES-1.6K_1%_0402:368 ↔ RES-1.6K_1%_0402:369
- Flush:1135: UND_0201CR___ _________:270 ↔ UND_0201CR___ _________:271
- Flush:1136: UND_0201CR___ _________:165 ↔ UND_0201CR___ _________:271
- [Flush]: RES-1.6K_1%_0402:372 ↔ RES-1.6K_1%_0402:373
- [Flush]: RES-1.6K_1%_0402:371 ↔ RES-1.6K_1%_0402:372
- Flush:1139: RES-1.6K_1%_0402:373 ↔ RES-1.6K_1%_0402:374
- Flush:1140: RES-1.6K_1%_0402:346 ↔ RES-1.6K_1%_0402:372
- Flush:1141: RES-1.6K_1%_0402:323 ↔ RES-1.6K_1%_0402:243
- Flush:1142: RES-1.6K_1%_0402:375 ↔ RES-1.6K_1%_0402:115
- Flush:1143: Cooling Kit for NVIDIA Jetson Xavier NX - screws-harness:1 ↔ P3767-pcba-envelop_20230310-modificada:1
- Mate:288: Cooling Kit for NVIDIA Jetson Xavier NX - screws-harness:1 ↔ P3767-pcba-envelop_20230310-modificada:1